# Autodesk Inventor assembly: Full Wheel Assembly
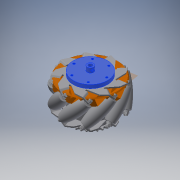
[picture p0: Inventor's stored thumbnail of the model, 180x180]
Saved by Autodesk Inventor 2017 (Build 210142000, 142)
## iProperties
Created: 2017-07-29
Part Number: Full Wheel Assembly
Document SubType Name: Assembly
Designer: User
Author: User
## Documents named in this file (5)
- C:\Robotics\CAD\2016-17_CAD\Full Wheel Assembly.iam
- C:\Robotics\CAD\COTSParts\Actobotics\615 parts\615114.ipt
- C:\Robotics\CAD\2016-17_CAD\Mecanum Wheel Adapter.ipt
- C:\Robotics\CAD\COTSParts\Wheels\AndyMark Mecanum Wheels\100mm Aluminum Mecanum wheels.ipt
- C:\Robotics\CAD\2016-17_CAD\Mecanum Wheel Adapter Plate.ipt
## Components (4 placed, 4 different names)
1. 615114:1 — Insert:1, Insert:2
2. Mecanum Wheel Adapter:1 — Insert:1, Insert:2, Insert:3, Insert:4, Insert:5
3. 100mm Aluminum Mecanum wheels:1 — Insert:3, Insert:4, Insert:6, Insert:7
4. Mecanum Wheel Adapter Plate:1 — Insert:5, Insert:6, Insert:7
## Relationships (7: Insert 7)
- Insert:1: 615114:1 ↔ Mecanum Wheel Adapter:1
- Insert:2: 615114:1 ↔ Mecanum Wheel Adapter:1
- Insert:3: Mecanum Wheel Adapter:1 ↔ 100mm Aluminum Mecanum wheels:1
- Insert:4: Mecanum Wheel Adapter:1 ↔ 100mm Aluminum Mecanum wheels:1
- Insert:5: Mecanum Wheel Adapter:1 ↔ Mecanum Wheel Adapter Plate:1
- Insert:6: 100mm Aluminum Mecanum wheels:1 ↔ Mecanum Wheel Adapter Plate:1
- Insert:7: 100mm Aluminum Mecanum wheels:1 ↔ Mecanum Wheel Adapter Plate:1
